# Autodesk Inventor assembly: Assembly_opentrons_microscope_slide_y
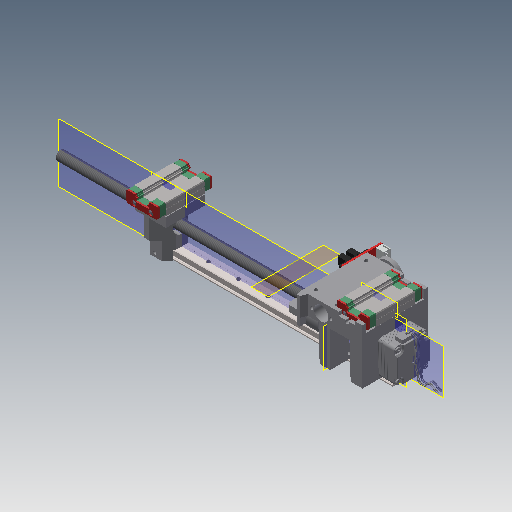
[picture p0: Inventor's stored thumbnail of the model, 512x512]
Saved by Autodesk Inventor 2019.4 (Build 234330000, 330)
## iProperties
Created: 2020-11-05
Part Number: Assembly_opentrons_microscope_slide_y
Document SubType Name: Assembly
Designer: diederichbenedict
Author: diederichbenedict
## Documents named in this file (11)
- C:\Users\diederichbenedict\Dropbox\Dokumente\Promotion\PROJECTS\OPENTRONS\INVENTOR\Assembly_opentrons_microscope_slide_y.iam
- C:\Users\diederichbenedict\Dropbox\Dokumente\Promotion\PROJECTS\OPENTRONS\INVENTOR\Assembly_spindeldrive_350mm.iam
- C:\Users\diederichbenedict\Dropbox\Dokumente\Promotion\PROJECTS\OPENTRONS\INVENTOR\01_Slide_camera_y_v0.ipt
- C:\Users\diederichbenedict\Dropbox\Dokumente\Promotion\PROJECTS\OPENTRONS\INVENTOR\00_NEMA11.iam
- C:\Users\diederichbenedict\Dropbox\Dokumente\Promotion\PROJECTS\OPENTRONS\INVENTOR\00_MGN12H, LINEAR GUIDE BLOCK.ipt
- C:\Users\diederichbenedict\Dropbox\Dokumente\Promotion\PROJECTS\OPENTRONS\INVENTOR\00_spindel_slide.ipt
- C:\Users\diederichbenedict\Dropbox\Dokumente\Promotion\PROJECTS\OPENTRONS\INVENTOR\03_Support_Xslide.ipt
- C:\Users\diederichbenedict\Dropbox\Dokumente\Promotion\PROJECTS\OPENTRONS\INVENTOR\00_endstop_optical.ipt
- C:\Users\diederichbenedict\Dropbox\Dokumente\Promotion\PROJECTS\OPENTRONS\INVENTOR\00_MGN12 LINEAR GUIDE RAIL, CONFIGURABLE.ipt
- C:\Users\diederichbenedict\Dropbox\Dokumente\Promotion\PROJECTS\OPENTRONS\INVENTOR\STL\04_Mount_Rail_Fastener.ipt
- C:\Users\diederichbenedict\Dropbox\Dokumente\Promotion\PROJECTS\OPENTRONS\INVENTOR\00_Endstop.ipt
## Components (11 placed, 10 different names)
1. 00_NEMA11:1 [sub-assembly]
2. Assembly_spindeldrive_350mm:1 [sub-assembly]
3. 01_Slide_camera_y_v0:1 — Flush:2, Insert:4, Mate:3, Mate:4, Flush:7, Insert:5, Angle:1, Flush:9
4. 00_MGN12H, LINEAR GUIDE BLOCK:1 — Flush:2
5. 00_spindel_slide:1 — Insert:4
6. 00_endstop_optical:1 — Mate:3, Mate:4, Flush:7
7. 00_MGN12H, LINEAR GUIDE BLOCK:2 — Flush:8
8. 00_Endstop:1 — Mate:13, Mate:14
9. 03_Support_Xslide:1 — Flush:8
10. 00_MGN12 LINEAR GUIDE RAIL, CONFIGURABLE:1 — Insert:5, Angle:1
11. 04_Mount_Rail_Fastener:1 — Flush:9, Mate:13, Mate:14
## Relationships (15: Flush 6, Mate 5, Insert 3, Angle 1)
- [Mate]: Assembly_spindeldrive_350mm:1 ↔ 01_Slide_camera_y_v0:1
- [Insert] (10 mm): 00_NEMA11:1 ↔ Assembly_spindeldrive_350mm:1
- Flush:2 (4.8 mm): 01_Slide_camera_y_v0:1 ↔ 00_MGN12H, LINEAR GUIDE BLOCK:1
- Insert:4: 01_Slide_camera_y_v0:1 ↔ 00_spindel_slide:1
- [Flush]: 00_MGN12H, LINEAR GUIDE BLOCK:1 ↔ 00_MGN12H, LINEAR GUIDE BLOCK:2
- Mate:3: 01_Slide_camera_y_v0:1 ↔ 00_endstop_optical:1
- Mate:4 (-20 mm): 01_Slide_camera_y_v0:1 ↔ 00_endstop_optical:1
- Flush:7: 01_Slide_camera_y_v0:1 ↔ 00_endstop_optical:1
- Flush:8: 00_MGN12H, LINEAR GUIDE BLOCK:2 ↔ 03_Support_Xslide:1
- Insert:5: 01_Slide_camera_y_v0:1 ↔ 00_MGN12 LINEAR GUIDE RAIL, CONFIGURABLE:1
- Angle:1 (0 deg): 01_Slide_camera_y_v0:1 ↔ 00_MGN12 LINEAR GUIDE RAIL, CONFIGURABLE:1
- Flush:9: 01_Slide_camera_y_v0:1 ↔ 04_Mount_Rail_Fastener:1
- [Flush] (3 mm): 00_Endstop:1 ↔ 04_Mount_Rail_Fastener:1
- Mate:13 (0.3 mm): 00_Endstop:1 ↔ 04_Mount_Rail_Fastener:1
- Mate:14 (1 mm): 00_Endstop:1 ↔ 04_Mount_Rail_Fastener:1
